# Autodesk Inventor assembly: Leg
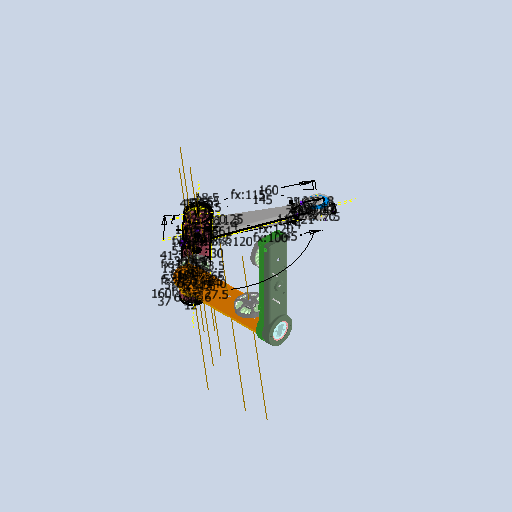
[picture p0: Inventor's stored thumbnail of the model, 512x512]
Saved by Autodesk Inventor 2023 (Build 270158000, 158)
## iProperties
Created: 2022-01-01
Part Number: Leg
Document SubType Name: Assembly
Designer: Jochen
Author: Jochen
## Documents named in this file (5)
- D:\Projects\Lisbeth\CAD\Leg Short.iam
- D:\Projects\Lisbeth\CAD\Thigh\Thigh.iam
- D:\Projects\Lisbeth\CAD\LowerLeg\LowerLeg.iam
- D:\Projects\Lisbeth\CAD\Hip\Hip Short.iam
- D:\Projects\Lisbeth\CAD\Lumbar\Lumbar Short.iam
## Components (4 placed, 4 different names)
1. Thigh:1 [sub-assembly] — Mate:5, Mate:12, Mate:13, Mate:15
2. LowerLeg:1 [sub-assembly] — Mate:12, Mate:13
3. Hip:1 [sub-assembly] — Mate:5, Mate:11, Mate:15, Mate:16
4. Lumbar:1 [sub-assembly] — Mate:11, Mate:16
## Relationships (6: Mate 6)
- Mate:5: Thigh:1 ↔ Hip:1
- Mate:11: Hip:1 ↔ Lumbar:1
- Mate:12: Thigh:1 ↔ LowerLeg:1
- Mate:13: Thigh:1 ↔ LowerLeg:1
- Mate:15: Thigh:1 ↔ Hip:1
- Mate:16: Hip:1 ↔ Lumbar:1
